# Autodesk Inventor assembly: Assembly2 стойка
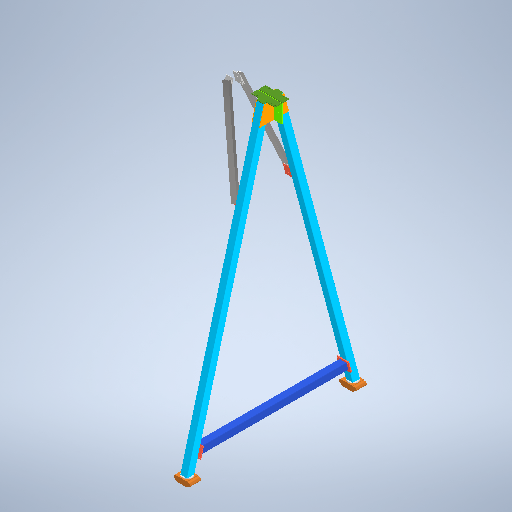
[picture p0: Inventor's stored thumbnail of the model, 512x512]
Saved by Autodesk Inventor 2025 (Build 290162010, 162A)
## iProperties
Created: 2024-06-18
Part Number: Assembly2 стойка
Document SubType Name: Assembly
Designer: admin
Author: admin
## Documents named in this file (12)
- C:\Users\pokla\Documents\Inventor\Goat 1\Assembly2 стойка.iam
- C:\Users\pokla\Documents\Inventor\Goat 1\Сrane plate 3.ipt
- C:\Users\pokla\Documents\Inventor\Goat 1\стойка 1 100x100x4 - 5000.ipt
- C:\Users\pokla\Documents\Inventor\Goat 1\Сrane plate 4.ipt
- C:\Users\pokla\Documents\Inventor\Goat 1\Сrane plate 6.ipt
- C:\Users\pokla\Documents\Inventor\Goat 1\Сrane plate 2.ipt
- C:\Users\pokla\Documents\Inventor\Goat 1\Сrane plate 5.ipt
- C:\Users\pokla\Documents\Inventor\Goat 1\roller platform.ipt
- C:\Users\pokla\Desktop\Г-образные закладные детали\Номенклатура Г-образных опор\foot.ipt
- C:\Users\pokla\Documents\Inventor\Goat 1\Сrane plate 5.1.ipt
- C:\Users\pokla\Documents\Inventor\Goat 1\JIS G 3192 - 100 x 50 x 5 - 1500 - 0,00936(4).ipt
- C:\Users\pokla\Desktop\Г-образные закладные детали\Номенклатура Г-образных опор\Стойка 2.ipt
## Components (29 placed, 17 different names)
1. Сrane plate 3.ipt:1 — Mate:11, Mate:12, Mate:13, Flush:6, Flush:7, Rigid:3
2. стойка 1 100x100x4 - 5000.ipt:1 — Mate:9, Mate:10, Rigid:1
3. Сrane plate 4.ipt:1
4. Сrane plate 6.ipt:1 — Rigid:7
5. Сrane plate 4.ipt:2
6. Сrane plate 2.ipt:1 — Mate:11, Mate:12, Mate:13
7. Сrane plate 5.ipt:1 — Mate:9, Mate:10, Rotational:2, Mate:25
8. roller platform:1 — Rigid:2, Mate:14
9. foot:1 — Rigid:1, Rigid:2
10. Сrane plate 5.1:1 — Rotational:2, Mate:25
11. JIS G 3192 - 100 x 50 x 5 - 1500 - 0,00936(4):1
12. Сrane plate 5.1:2
13. Сrane plate 5:2
14. Сrane plate 3:2 — Rigid:3, Rigid:4, Mate:18, Mate:20
15. Сrane plate 2:2 — Rigid:4, Mate:19, Mate:21, Mate:23
16. Сrane plate 4:3 — Mate:18, Mate:19, Flush:12, Flush:13
17. Сrane plate 4:4 — Mate:20, Mate:21, Mate:22, Mate:24
18. стойка 1 100x100x4 - 5000:2 — Mate:23, Mate:24, Flush:13, Rigid:5, Mate:26, Mate:29, Flush:31, Mate:35, Mate:38
19. foot:2 — Rigid:5, Rigid:6
20. roller platform:2 — Rigid:6
21. Сrane plate 6:2 — Mate:26, Mate:27, Rigid:8, Mate:38
22. Сrane plate 5:3 — Mate:29, Flush:31, Mate:35, Rotational:4, Mate:36
23. Сrane plate 5.1:3 — Rotational:4, Mate:36
24. JIS G 3192 - 100 x 50 x 5 - 1500 - 0,00936(4):2
25. Сrane plate 5.1:4 — Rotational:5, Mate:37
26. Сrane plate 5:4 — Rotational:5, Mate:37
27. Сrane plate 6:3 — Rigid:7
28. Сrane plate 6:4 — Rigid:8, Mate:41
29. Стойка 2:1 — Mate:39, Mate:40, Mate:41
## Relationships (67: Mate 37, Flush 18, WeldJoint 8, RevoluteJoint 4)
- [Mate]: стойка 1 100x100x4 - 5000.ipt:1 ↔ Сrane plate 4.ipt:1
- [Mate]: стойка 1 100x100x4 - 5000.ipt:1 ↔ Сrane plate 4.ipt:2
- [Flush]: стойка 1 100x100x4 - 5000.ipt:1 ↔ Сrane plate 4.ipt:2
- [Flush]: стойка 1 100x100x4 - 5000.ipt:1 ↔ Сrane plate 4.ipt:1
- [Flush]: стойка 1 100x100x4 - 5000.ipt:1 ↔ Сrane plate 4.ipt:1
- [Flush]: стойка 1 100x100x4 - 5000.ipt:1 ↔ Сrane plate 4.ipt:2
- [Flush]: стойка 1 100x100x4 - 5000.ipt:1 ↔ Сrane plate 2.ipt:1
- [Mate]: стойка 1 100x100x4 - 5000.ipt:1 ↔ Сrane plate 2.ipt:1
- [Mate]: стойка 1 100x100x4 - 5000.ipt:1 ↔ Сrane plate 6.ipt:1
- [Mate]: стойка 1 100x100x4 - 5000.ipt:1 ↔ Сrane plate 6.ipt:1
- [Mate]: Сrane plate 3.ipt:1 ↔ Сrane plate 4.ipt:2
- [Mate] (-200 mm): стойка 1 100x100x4 - 5000.ipt:1 ↔ Сrane plate 6.ipt:1
- [Mate]: стойка 1 100x100x4 - 5000.ipt:1 ↔ Сrane plate 5.ipt:1
- Mate:9 (-45 mm): стойка 1 100x100x4 - 5000.ipt:1 ↔ Сrane plate 5.ipt:1
- Mate:10 (1272 mm): стойка 1 100x100x4 - 5000.ipt:1 ↔ Сrane plate 5.ipt:1
- Mate:11: Сrane plate 3.ipt:1 ↔ Сrane plate 2.ipt:1
- Mate:12: Сrane plate 3.ipt:1 ↔ Сrane plate 2.ipt:1
- Mate:13: Сrane plate 3.ipt:1 ↔ Сrane plate 2.ipt:1
- Flush:6: Сrane plate 3.ipt:1
- Flush:7: Сrane plate 3.ipt:1
- Rigid:1 [WeldJoint]: стойка 1 100x100x4 - 5000.ipt:1 ↔ foot:1
- Rigid:2 [WeldJoint]: roller platform:1 ↔ foot:1
- Mate:14: roller platform:1
- [Flush]: Сrane plate 5.1:1 ↔ JIS G 3192 - 100 x 50 x 5 - 1500 - 0,00936(4):1
- [Flush]: Сrane plate 5.1:1 ↔ JIS G 3192 - 100 x 50 x 5 - 1500 - 0,00936(4):1
- [Mate]: Сrane plate 5.1:1 ↔ JIS G 3192 - 100 x 50 x 5 - 1500 - 0,00936(4):1
- [Flush]: JIS G 3192 - 100 x 50 x 5 - 1500 - 0,00936(4):1 ↔ Сrane plate 5.1:2
- [Flush]: JIS G 3192 - 100 x 50 x 5 - 1500 - 0,00936(4):1 ↔ Сrane plate 5.1:2
- [Mate]: JIS G 3192 - 100 x 50 x 5 - 1500 - 0,00936(4):1 ↔ Сrane plate 5.1:2
- [RevoluteJoint]: Сrane plate 5.1:2 ↔ Сrane plate 5:2
- [Mate]: Сrane plate 5.1:2 ↔ Сrane plate 5:2
- Rotational:2 [RevoluteJoint]: Сrane plate 5.ipt:1 ↔ Сrane plate 5.1:1
- Rigid:3 [WeldJoint]: Сrane plate 3.ipt:1 ↔ Сrane plate 3:2
- Rigid:4 [WeldJoint]: Сrane plate 3:2 ↔ Сrane plate 2:2
- Mate:18: Сrane plate 3:2 ↔ Сrane plate 4:3
- Mate:19: Сrane plate 2:2 ↔ Сrane plate 4:3
- Flush:12 (60 mm): Сrane plate 4:3
- Mate:20: Сrane plate 3:2 ↔ Сrane plate 4:4
- Mate:21: Сrane plate 2:2 ↔ Сrane plate 4:4
- Mate:22 (60 mm): Сrane plate 4:4
- Mate:23: Сrane plate 2:2 ↔ стойка 1 100x100x4 - 5000:2
- Mate:24: Сrane plate 4:4 ↔ стойка 1 100x100x4 - 5000:2
- Flush:13: Сrane plate 4:3 ↔ стойка 1 100x100x4 - 5000:2
- Rigid:5 [WeldJoint]: стойка 1 100x100x4 - 5000:2 ↔ foot:2
- Rigid:6 [WeldJoint]: foot:2 ↔ roller platform:2
- Mate:25: Сrane plate 5.ipt:1 ↔ Сrane plate 5.1:1
- Mate:26: стойка 1 100x100x4 - 5000:2 ↔ Сrane plate 6:2
- Mate:27: Сrane plate 6:2
- Mate:29: стойка 1 100x100x4 - 5000:2 ↔ Сrane plate 5:3
- Flush:31 (45 mm): стойка 1 100x100x4 - 5000:2 ↔ Сrane plate 5:3
- [Flush]: Сrane plate 5.1:3 ↔ JIS G 3192 - 100 x 50 x 5 - 1500 - 0,00936(4):2
- [Flush]: Сrane plate 5.1:3 ↔ JIS G 3192 - 100 x 50 x 5 - 1500 - 0,00936(4):2
- [Mate]: Сrane plate 5.1:3 ↔ JIS G 3192 - 100 x 50 x 5 - 1500 - 0,00936(4):2
- [Flush]: JIS G 3192 - 100 x 50 x 5 - 1500 - 0,00936(4):2 ↔ Сrane plate 5.1:4
- [Flush]: JIS G 3192 - 100 x 50 x 5 - 1500 - 0,00936(4):2 ↔ Сrane plate 5.1:4
- [Mate]: JIS G 3192 - 100 x 50 x 5 - 1500 - 0,00936(4):2 ↔ Сrane plate 5.1:4
- Mate:35 (1270 mm): стойка 1 100x100x4 - 5000:2 ↔ Сrane plate 5:3
- Rotational:4 [RevoluteJoint]: Сrane plate 5:3 ↔ Сrane plate 5.1:3
- Mate:36: Сrane plate 5:3 ↔ Сrane plate 5.1:3
- Rotational:5 [RevoluteJoint]: Сrane plate 5.1:4 ↔ Сrane plate 5:4
- Mate:37: Сrane plate 5.1:4 ↔ Сrane plate 5:4
- Rigid:7 [WeldJoint]: Сrane plate 6.ipt:1 ↔ Сrane plate 6:3
- Rigid:8 [WeldJoint]: Сrane plate 6:2 ↔ Сrane plate 6:4
- Mate:38 (-200 mm): стойка 1 100x100x4 - 5000:2 ↔ Сrane plate 6:2
- Mate:39: Стойка 2:1
- Mate:40: Стойка 2:1
- Mate:41 (26.8 mm): Сrane plate 6:4 ↔ Стойка 2:1
## Named parameters: d52_d65 = 0 mm, d53_d66 = 0 mm, d54_d67 = 0 mm, d55_d68 = 0 mm, d96_d52_d65 = 0 mm, d97_d53_d66 = 0 mm, d98_d54_d67 = 0 mm, d99_d55_d68 = 0 mm, d100_d69 = 0 mm, d101_d70 = 0 mm
